# Autodesk Inventor assembly: Assy_foot
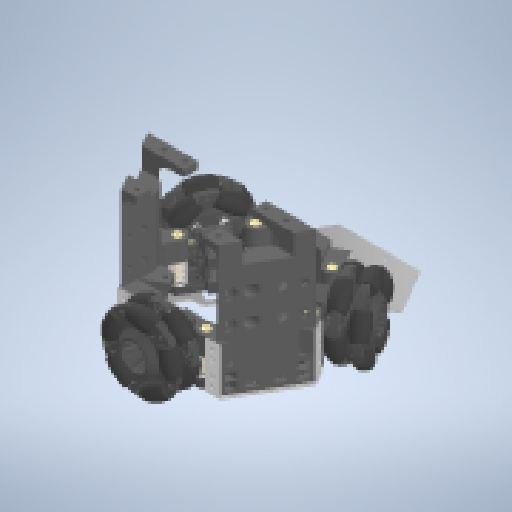
[picture p0: Inventor's stored thumbnail of the model, 512x512]
Saved by Autodesk Inventor 2024.1 (Build 281209000, 209)
## iProperties
Created: 2025-02-03
Part Number: Assy_foot
Document SubType Name: Assembly
Designer: hibik
Author: hibik
## Documents named in this file (3)
- C:\Users\hibik\Documents\Robomech\RESCUE\ORCA\hard\Assy_foot.iam
- C:\Users\hibik\Documents\Robomech\RESCUE\ORCA\hard\flame_base\base.iam
- C:\Users\hibik\Documents\Robomech\RESCUE\ORCA\hard\omni_wheel\Assy_omni_wheel.iam
## Components (4 placed, 2 different names)
1. base:1 [sub-assembly] — 挿入:5, 挿入:6, 挿入:7, 挿入:8, 挿入:9, 挿入:10
2. Assy_omni_wheel:3 [sub-assembly] — 挿入:5, 挿入:6
3. Assy_omni_wheel:4 [sub-assembly] — 挿入:7, 挿入:8
4. Assy_omni_wheel:5 [sub-assembly] — 挿入:9, 挿入:10
## Relationships (6: Insert 6)
- 挿入:5 [Insert]: base:1 ↔ Assy_omni_wheel:3
- 挿入:6 [Insert]: base:1 ↔ Assy_omni_wheel:3
- 挿入:7 [Insert]: base:1 ↔ Assy_omni_wheel:4
- 挿入:8 [Insert]: base:1 ↔ Assy_omni_wheel:4
- 挿入:9 [Insert]: base:1 ↔ Assy_omni_wheel:5
- 挿入:10 [Insert]: base:1 ↔ Assy_omni_wheel:5
